# Autodesk Inventor assembly: battery terminal presentation
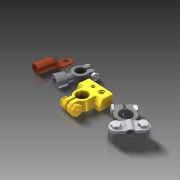
[picture p0: Inventor's stored thumbnail of the model, 180x180]
Saved by Autodesk Inventor 2014 (Build 180170000, 170)
## iProperties
Created: 2013-07-25
Part Number: battery terminal presentation
Document SubType Name: Assembly
Designer: Saville
Mass: 42.4824 g
Surface Area: 265.422 cm^2
Volume: 42.4824 cm^3
Density: 1 g/cm^3
Author: Saville
## Documents named in this file (5)
- C:\electrical nuts\terminal\battery terminal presentation.iam
- C:\electrical nuts\terminal\sae terminal tube style\sae terminal tube style.ipt
- C:\electrical nuts\terminal\multi battery terminal\battery terminal.ipt
- C:\electrical nuts\terminal\copper solder battery terminal\copper battery terminal.ipt
- C:\electrical nuts\terminal\battery terminal1\sea terminal.ipt
## Components (4 placed, 4 different names)
1. sae terminal tube style:1 — Mate:3
2. battery terminal:1 — Mate:1
3. copper battery terminal:1 — Mate:4
4. sea terminal:1 — Mate:2
## Relationships (4: Mate 4)
- Mate:1: battery terminal:1
- Mate:2: sea terminal:1
- Mate:3: sae terminal tube style:1
- Mate:4: copper battery terminal:1
